# Autodesk Inventor assembly: Drive Roller Assembly 3 (Lexan)
(part 2 of 2)
- Mate:1152: Hex Shaft 1-2 in (am-0856):2 ↔ Hex Shaft Connector (Lexan):4
- Mate:1153 (38.1 mm): Lexan flexible Arm Mount:1 ↔ Lexan flexible Arm Mount:2
- Mate:1154 (38.1 mm): Lexan flexible Arm Mount:3 ↔ Lexan flexible Arm Mount:4
- Flush:31: Hex Shaft 1-2 in (am-0856):2 ↔ Hex Shaft Collar 1-2 in (7552K500):19
- Mate:1155: Pneumatic Piston Front Flange (Rt Custom):2 ↔ Clamp with Piston Assembly (new):1
- Mate:1156: Pneumatic Piston Front Flange (Rt Custom):2 ↔ Clamp with Piston Assembly (new):1
- Mate:1157: Pneumatic Piston Front Flange (Rt Custom):2 ↔ Clamp with Piston Assembly (new):1
- Mate:1159: Hex Shaft Collar 3-8 in (7552K300):4 ↔ Clamp with Piston Assembly (new):1
- Mate:1160: Pneumatic Piston Front Flange (Lt Custom):1 ↔ Clamp with Piston Assembly (new):2
- Mate:1161: Pneumatic Piston Front Flange (Lt Custom):1 ↔ Clamp with Piston Assembly (new):2
- Mate:1162: Pneumatic Piston Front Flange (Lt Custom):1 ↔ Clamp with Piston Assembly (new):2
- Mate:1163: Hex Shaft Collar 3-8 in (7552K300):1 ↔ Clamp with Piston Assembly (new):2
- Mate:1164: Hex Shaft Collar 3-8 in (7552K300):2 ↔ Clamp with Piston Assembly (new):2
- Flush:32: Hex Shaft 3-8 in (am-0855):1 ↔ Hex Shaft Collar 3-8 in (7552K300):2
- Flush:33 (-15.875 mm): Hex Shaft 3-8 in (am-0855):1 ↔ Hex Spacer:7
- Mate:1165: Hex Shaft Collar 3-8 in (7552K300):6 ↔ Clamp with Piston Assembly (new):2
- Mate:1166: Hex Shaft Collar 3-8 in (7552K300):7 ↔ Clamp with Piston Assembly (new):2
- Mate:1167: Hex Shaft Collar 3-8 in (7552K300):1 ↔ Clamp with Piston Assembly (new):2
- Flush:34: Hex Shaft 3-8 in (am-0855):2 ↔ Hex Shaft Collar 3-8 in (7552K300):4
- Mate:1168: Hex Shaft Collar 3-8 in (7552K300):8 ↔ Clamp with Piston Assembly (new):1
- Mate:1169: Hex Shaft Collar 3-8 in (7552K300):5 ↔ Clamp with Piston Assembly (new):1
- Mate:1170: Hex Shaft Collar 3-8 in (7552K300):3 ↔ Clamp with Piston Assembly (new):1
- Mate:1172: Vex Pro 1x1 rectangular tubing 14 in length:5 ↔ Roller Piston 4 (.5 and 1 in Stroke, 9-16 in Bore):3
- Mate:1173: Vex Pro 1x1 rectangular tubing 14 in length:5 ↔ Roller Piston 4 (.5 and 1 in Stroke, 9-16 in Bore):3
- Mate:1174: Vex Pro 1x1 rectangular tubing 14 in length:5 ↔ Roller Piston 4 (.5 and 1 in Stroke, 9-16 in Bore):3
- Mate:1175: Bracket:2 ↔ Roller Piston 4 (.5 and 1 in Stroke, 9-16 in Bore):3
- Mate:1176: Shaft Collar 3-16 in ID (6435K510):2 ↔ Roller Piston 4 (.5 and 1 in Stroke, 9-16 in Bore):3
- Mate:1177: Shaft Collar 3-16 in ID (6435K510):1 ↔ Roller Piston 4 (.5 and 1 in Stroke, 9-16 in Bore):3
- Mate:1178: Vex Pro 1x1 rectangular tubing 14 in length:6 ↔ Roller Piston 4 (.5 and 1 in Stroke, 9-16 in Bore):2
- Mate:1179: Vex Pro 1x1 rectangular tubing 14 in length:6 ↔ Roller Piston 4 (.5 and 1 in Stroke, 9-16 in Bore):2
- Mate:1180: Bracket:4 ↔ Roller Piston 4 (.5 and 1 in Stroke, 9-16 in Bore):2
- Mate:1181: Shaft Collar 3-16 in ID (6435K510):3 ↔ Roller Piston 4 (.5 and 1 in Stroke, 9-16 in Bore):2
- Mate:1182: Shaft Collar 3-16 in ID (6435K510):4 ↔ Roller Piston 4 (.5 and 1 in Stroke, 9-16 in Bore):2
- Mate:1183: Hex Shaft Collar 3-8 in (7552K300):3 ↔ Clamp with Piston Assembly (new):1
- Mate:1184: Vex Pro 1x1 rectangular tubing 14 in length:5 ↔ Vex Pro T gusset - OUT OF STOCK 1192014:1
- Mate:1185: Vex Pro 1x1 rectangular tubing 14 in length:5 ↔ Vex Pro T gusset - OUT OF STOCK 1192014:1
- Mate:1186: Vex Pro 1x1 rectangular tubing 14 in length:5 ↔ Vex Pro T gusset - OUT OF STOCK 1192014:1
- Mate:1187: Vex Pro 1x1 rectangular tubing 4 in length:3 ↔ Vex Pro T gusset - OUT OF STOCK 1192014:1
- Flush:35: Vex Pro 1x1 rectangular tubing 4 in length:3 ↔ Vex Pro T gusset - OUT OF STOCK 1192014:1
- Mate:1188: Vex Pro T gusset - OUT OF STOCK 1192014:1 ↔ Vex Pro 1x1 rectangular tubing 2 in length (no hex):1
- Mate:1189: Vex Pro T gusset - OUT OF STOCK 1192014:1 ↔ Vex Pro 1x1 rectangular tubing 2 in length (no hex):1
- Flush:36: Vex Pro T gusset - OUT OF STOCK 1192014:1 ↔ Vex Pro 1x1 rectangular tubing 2 in length (no hex):1
- Mate:1190: Vex Pro 1x1 rectangular tubing 14 in length:5 ↔ Vex Pro T gusset - OUT OF STOCK 1192014:2
- Mate:1191: Vex Pro 1x1 rectangular tubing 14 in length:5 ↔ Vex Pro T gusset - OUT OF STOCK 1192014:2
- Mate:1192: Vex Pro 1x1 rectangular tubing 14 in length:5 ↔ Vex Pro T gusset - OUT OF STOCK 1192014:2
- Mate:1193: Vex Pro 1x1 rectangular tubing 2 in length (no hex):1 ↔ Vex Pro T gusset - OUT OF STOCK 1192014:2
- Mate:1194: Vex Pro 1x1 rectangular tubing 4 in length:3 ↔ Vex Pro T gusset - OUT OF STOCK 1192014:2
- Mate:1195: Vex Pro 1x1 rectangular tubing 14 in length (roller):1 ↔ Roller Crossbar Gusset (Custom):5
- Mate:1196: Vex Pro 1x1 rectangular tubing 14 in length (roller):1 ↔ Roller Crossbar Gusset (Custom):5
- Mate:1197: Vex Pro 1x1 rectangular tubing 14 in length (roller):2 ↔ Roller Crossbar Gusset (Custom):4
- Mate:1198: Vex Pro 1x1 rectangular tubing 14 in length (roller):2 ↔ Roller Crossbar Gusset (Custom):4
## Named parameters: d240_d195 = 0 mm, d241_d196 = 0 mm, d242_d197 = 0 mm, d243_d198 = 0 mm, d305_d302 = 0 mm, d306_d303 = 0 mm, d307_d304 = 0 mm, d334_d317 = 0 mm, d335_d318 = -19.05 mm, d339_d304 = 0 mm, d343_d308 = 0 mm, d344_d309 = 0 mm, d345_d310 = 0 mm, d346_d316 = 0 mm, d349_d328 = 0 mm, d350_d329 = 0 mm, d352_d331 = 0 mm, d353_d332 = 0 mm, d770_d743 = 0 mm, d771_d744 = 0 mm, d772_d745 = 0 mm, d773_d746 = 0 mm, d791_d742 = 0 mm, d1331_d1327 = 0 mm, d1332_d1328 = 0 mm, d1398_d1387 = 0 mm, d1399_d1388 = 0 mm, d1400_d1389 = 0 mm, d1404_d1384 = 0 mm, d1405_d1385 = 0 mm, d1406_d1386 = 0 mm
